# Autodesk Inventor assembly: Nema17
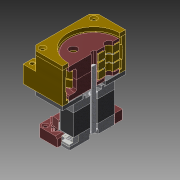
[picture p0: Inventor's stored thumbnail of the model, 180x180]
Saved by Autodesk Inventor 2022 (Build 260153000, 153)
## iProperties
Part Number: Nema17
Checked By: Якушев
Engr Approved By: Малов
Material: Типовые
Document SubType Name: Assembly
Mfg Approved By: Судаков
Designer: Смирнов
Author: Смирнов
## Documents named in this file (9)
- C:\Школа\1517_Предпроф_2024-2025\Наливатор_акт\Shoter_1_ZIP\Nema17.iam
- C:\Школа\1517_Предпроф_2024-2025\Наливатор_акт\Shoter_1_ZIP\Pumpshare.iam
- C:\Школа\1517_Предпроф_2024-2025\Наливатор_акт\Shoter_1_ZIP\Abec 7 608 zz.ipt
- C:\Школа\1517_Предпроф_2024-2025\Наливатор_акт\Shoter_1_ZIP\Полумуфта.ipt
- C:\Школа\1517_Предпроф_2024-2025\Наливатор_акт\Shoter_1_ZIP\Втулка.ipt
- C:\Школа\1517_Предпроф_2024-2025\Наливатор_акт\Shoter_1_ZIP\Корпус.ipt
- C:\Школа\1517_Предпроф_2024-2025\Наливатор_акт\Shoter_1_ZIP\Крышка.ipt
- C:\Школа\1517_Предпроф_2024-2025\Наливатор_акт\Shoter_1_ZIP\Держатель.ipt
- C:\Школа\1517_Предпроф_2024-2025\Наливатор_акт\Shoter_1_ZIP\Насос_Основание_нижнее.ipt
## Components (21 placed, 8 different names)
1. NEMA17 [sub-assembly] — Заподлицо:5
2. Насос Основание_нижнее:1
3. Полумуфта:1 — Совмещение:1, Совмещение:2, Совмещение:4, Совмещение:5
4. Корпус:1 — Заподлицо:4
5. Крышка:1 — Заподлицо:4
6. Держатель:1 — Заподлицо:5
7. Abec 7 608 zz:5 — Совмещение:9
8. Abec 7 608 zz:4 — Совмещение:2, Совмещение:3, Совмещение:4, Совмещение:6
9. Abec 7 608 zz:1 — Совмещение:1, Совмещение:5, Совмещение:9, Совмещение:10
10. Втулка:1 — Совмещение:3, Совмещение:6
11. Втулка:2 — Совмещение:10
12. Abec 7 608 zz:6
13. Abec 7 608 zz:7
14. Abec 7 608 zz:8
15. Втулка:3
16. Втулка:4
17. Abec 7 608 zz:9
18. Abec 7 608 zz:10
19. Abec 7 608 zz:11
20. Втулка:5
21. Втулка:6
## Component patterns: (3 elements, first: Abec 7 608 zz:5 + Abec 7 608 zz:4 + Abec 7 608 zz:1 + Втулка:1 + Втулка:2)
## Relationships (14: Mate 10, Flush 4)
- [Flush]: Насос Основание_нижнее:1 ↔ Полумуфта:1
- Совмещение:1 [Mate]: Полумуфта:1 ↔ Abec 7 608 zz:1
- Совмещение:2 [Mate]: Полумуфта:1 ↔ Abec 7 608 zz:4
- Совмещение:3 [Mate]: Abec 7 608 zz:4 ↔ Втулка:1
- Совмещение:4 [Mate]: Полумуфта:1 ↔ Abec 7 608 zz:4
- Совмещение:5 [Mate]: Полумуфта:1 ↔ Abec 7 608 zz:1
- Совмещение:6 [Mate]: Abec 7 608 zz:4 ↔ Втулка:1
- [Flush]: Насос Основание_нижнее:1 ↔ Корпус:1
- Заподлицо:4 [Flush]: Корпус:1 ↔ Крышка:1
- [Mate]: Abec 7 608 zz:5 ↔ Втулка:2
- [Mate]: Abec 7 608 zz:5 ↔ Втулка:2
- Совмещение:9 [Mate]: Abec 7 608 zz:5 ↔ Abec 7 608 zz:1
- Совмещение:10 [Mate]: Abec 7 608 zz:1 ↔ Втулка:2
- Заподлицо:5 [Flush]: NEMA17 ↔ Держатель:1
## Named parameters: d12_d7 = 0 mm, d13_d4 = 0 mm
